# Autodesk Inventor assembly: WheelAssembly
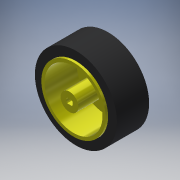
[picture p0: Inventor's stored thumbnail of the model, 180x180]
Saved by Autodesk Inventor 2018 (Build 220112000, 112)
## iProperties
Created: 2018-01-12
Part Number: WheelAssembly
Document SubType Name: Assembly
Designer: Kyle
Author: Kyle
## Documents named in this file (3)
- B:\My Documents\Project documentation\Hackathon-2018\Inventor\Robot\WheelAssembly.iam
- B:\My Documents\Project documentation\Hackathon-2018\Inventor\Robot\Wheel.ipt
- B:\My Documents\Project documentation\Hackathon-2018\Inventor\Robot\Tire.ipt
## Components (2 placed, 2 different names)
1. Wheel:1 — Mate:1, Flush:1
2. Tire:1 — Mate:1, Flush:1
## Relationships (2: Mate 1, Flush 1)
- Mate:1: Wheel:1 ↔ Tire:1
- Flush:1 (1.905 mm): Wheel:1 ↔ Tire:1
